# Autodesk Inventor assembly: Leg Assembly
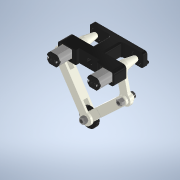
[picture p0: Inventor's stored thumbnail of the model, 180x180]
Saved by Autodesk Inventor 2022 (Build 260153000, 153)
## iProperties
Created: 2021-11-22
Part Number: Leg Assembly
Document SubType Name: Assembly
Designer: JK
Author: JK
## Documents named in this file (5)
- C:\Users\JK\Documents\Inventor\N20 Leg Actuator\N20-Leg-Actuator\CADfiles\Leg Assembly (small bearing).iam
- C:\Users\JK\Documents\Inventor\N20 Leg Actuator\N20-Leg-Actuator\CADfiles\Brushed DC Motor v8.iam
- C:\Users\JK\Documents\Inventor\N20 Leg Actuator\N20-Leg-Actuator\CADfiles\LegLinksAssembly.iam
- C:\Users\JK\Documents\Inventor\N20 Leg Actuator\N20-Leg-Actuator\CADfiles\ServoPot.ipt
- C:\Users\JK\Documents\Inventor\N20 Leg Actuator\N20-Leg-Actuator\CADfiles\Chasis.iam
## Components (6 placed, 4 different names)
1. Brushed DC Motor v8:1 [sub-assembly] — Coincidencia:48
2. Brushed DC Motor v8:2 [sub-assembly] — Coincidencia:49
3. LegLinksAssembly:1 [sub-assembly] — Coincidencia:43, Coincidencia:44, Coincidencia:45, Coincidencia:48, Coincidencia:49
4. ServoPot:1 — Coincidencia:43, Coincidencia:44, Nivelación:19
5. ServoPot:2 — Coincidencia:45, Nivelación:19, Nivelación:21
6. Chasis:1 [sub-assembly] — Coincidencia:47, Nivelación:20, Nivelación:21
## Relationships (15: Mate 10, Flush 3, Angle 2)
- [Mate]: Brushed DC Motor v8:1 ↔ Chasis:1
- [Mate]: Brushed DC Motor v8:1 ↔ Chasis:1
- [Angle] (0 deg): Brushed DC Motor v8:1 ↔ Chasis:1
- [Mate]: Brushed DC Motor v8:2 ↔ Chasis:1
- [Angle] (0 deg): Brushed DC Motor v8:2 ↔ Chasis:1
- [Mate]: Brushed DC Motor v8:2 ↔ Chasis:1
- Coincidencia:43 [Mate]: LegLinksAssembly:1 ↔ ServoPot:1
- Coincidencia:44 [Mate]: LegLinksAssembly:1 ↔ ServoPot:1
- Coincidencia:45 [Mate]: LegLinksAssembly:1 ↔ ServoPot:2
- Nivelación:19 [Flush]: ServoPot:1 ↔ ServoPot:2
- Coincidencia:47 [Mate]: Chasis:1
- Nivelación:20 [Flush]: Chasis:1
- Coincidencia:48 [Mate]: Brushed DC Motor v8:1 ↔ LegLinksAssembly:1
- Coincidencia:49 [Mate]: Brushed DC Motor v8:2 ↔ LegLinksAssembly:1
- Nivelación:21 [Flush] (-0.5 mm): ServoPot:2 ↔ Chasis:1
